# Autodesk Inventor assembly: WeaponAndMount
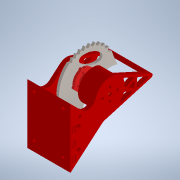
[picture p0: Inventor's stored thumbnail of the model, 180x180]
Saved by Autodesk Inventor 2020 (Build 240168000, 168)
## iProperties
Created: 2024-02-19
Part Number: WeaponAndMount
Document SubType Name: Assembly
Designer: smz3rm
Mass: 165.241 g
Surface Area: 469.895 cm^2
Volume: 71.0962 cm^3
Density: 2.32419 g/cm^3
Author: smz3rm
## Documents named in this file (3)
- C:\Users\smz3rm\OneDrive - BP\Documents\Battlebots\VerticalSpinner\WeaponAndMount.iam
- C:\Users\smz3rm\OneDrive - BP\Documents\Battlebots\VerticalSpinner\VertWeaponMount.iam
- C:\Users\smz3rm\OneDrive - BP\Documents\Battlebots\VerticalSpinner\WeaponAssembly.iam
## Components (2 placed, 2 different names)
1. VertWeaponMount:1 [sub-assembly] — Mate:1, Mate:2, Mate:3
2. WeaponAssembly:1 [sub-assembly] — Mate:1, Mate:2, Mate:3
## Relationships (3: Mate 3)
- Mate:1: VertWeaponMount:1 ↔ WeaponAssembly:1
- Mate:2: VertWeaponMount:1 ↔ WeaponAssembly:1
- Mate:3: VertWeaponMount:1 ↔ WeaponAssembly:1
